# Autodesk Inventor assembly: Assembly1
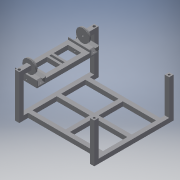
[picture p0: Inventor's stored thumbnail of the model, 180x180]
Saved by Autodesk Inventor 2018 (Build 220112000, 112)
## iProperties
Created: 2017-08-14
Part Number: Assembly1
Document SubType Name: Assembly
Designer: andre
Author: andre
## Documents named in this file (5)
- E:\Dropbox\AarhusUNI\Andet 2017\OrbitRaket\Assembly1.iam
- E:\Dropbox\AarhusUNI\Andet 2017\OrbitRaket\Raket_Arme.ipt
- E:\Dropbox\AarhusUNI\Andet 2017\OrbitRaket\Raket_Hjul.ipt
- E:\Dropbox\AarhusUNI\Andet 2017\OrbitRaket\Raket_Holder.ipt
- E:\Dropbox\AarhusUNI\Andet 2017\OrbitRaket\Raket_Lednings_Holder.ipt
## Components (6 placed, 4 different names)
1. Raket_Arme:1 — Rotational:7, Rigid:3, Rotational:9, Rotational:11
2. Raket_Holder:1 — Rotational:8, Rotational:9
3. Raket_Lednings_Holder:1
4. Raket_Arme:4 — Rotational:6, Rotational:8, Rotational:10
5. Raket_Hjul:2 — Rotational:6, Rotational:11
6. Raket_Hjul:3 — Rotational:7, Rigid:3, Rotational:10
## Relationships (7: RevoluteJoint 6, WeldJoint 1)
- Rotational:6 [RevoluteJoint]: Raket_Arme:4 ↔ Raket_Hjul:2
- Rotational:7 [RevoluteJoint]: Raket_Arme:1 ↔ Raket_Hjul:3
- Rigid:3 [WeldJoint]: Raket_Arme:1 ↔ Raket_Hjul:3
- Rotational:8 [RevoluteJoint]: Raket_Holder:1 ↔ Raket_Arme:4
- Rotational:9 [RevoluteJoint]: Raket_Arme:1 ↔ Raket_Holder:1
- Rotational:10 [RevoluteJoint]: Raket_Arme:4 ↔ Raket_Hjul:3
- Rotational:11 [RevoluteJoint]: Raket_Arme:1 ↔ Raket_Hjul:2
